# Autodesk Inventor assembly: Motor_28
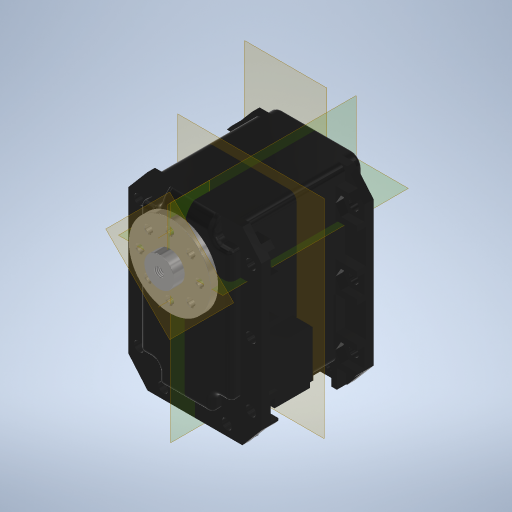
[picture p0: Inventor's stored thumbnail of the model, 512x512]
Saved by Autodesk Inventor 2024.3 (Build 283343000, 343)
## iProperties
Created: 2024-09-05
Part Number: Motor_28
Document SubType Name: Assembly
Designer: gretc
Author: gretc
## Documents named in this file (3)
- C:\Users\gretc\Desktop\inventor_part\Motor_28.iam
- C:\Users\gretc\Desktop\inventor_part\다이나믹셀\MX-28T_R_MIR.ipt
- C:\Users\gretc\Desktop\inventor_part\혼\28Horn.ipt
## Components (2 placed, 2 different names)
1. MX-28T_R_MIR:1 — 삽입:1, 각도:1
2. 28Horn:1 — 삽입:1, 메이트:1, 메이트:2
## Relationships (6: Mate 4, Insert 1, Angle 1)
- 삽입:1 [Insert] (0.5 mm): MX-28T_R_MIR:1 ↔ 28Horn:1
- 메이트:1 [Mate]: 28Horn:1
- 메이트:2 [Mate]: 28Horn:1
- 메이트:3 [Mate]
- 메이트:4 [Mate]
- 각도:1 [Angle] (90 deg): MX-28T_R_MIR:1
